# Autodesk Inventor assembly: populated-keyboard_cherrymx
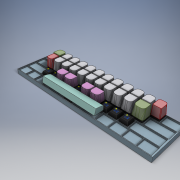
[picture p0: Inventor's stored thumbnail of the model, 180x180]
Saved by Autodesk Inventor 2016 (Build 200138000, 138)
## iProperties
Created: 2016-12-08
Part Number: populated-keyboard_cherrymx
Document SubType Name: Assembly
Designer: Cemra JC
Author: Cemra JC
## Documents named in this file (10)
- J:\The Files\The Software Files\Projects\stenotoppers\cherrymx\base-model\populated-keyboard_cherrymx.iam
- J:\The Files\The Software Files\Projects\stenotoppers\cherrymx\base-model\keyboard-mockup_cherrymx.iam
- J:\The Files\The Software Files\Projects\stenotoppers\cherrymx\base-model\standard-keycap_top-rows_base_cherrymx.ipt
- J:\The Files\The Software Files\Projects\stenotoppers\cherrymx\base-model\keyswitch_cherrymx.iam
- J:\The Files\The Software Files\Projects\stenotoppers\cherrymx\base-model\spacebar-keycap_mockup_cherrymx.ipt
- J:\The Files\The Software Files\Projects\stenotoppers\cherrymx\base-model\thumb-keycap_thumb-row_base_cherrymx.ipt
- J:\The Files\The Software Files\Projects\stenotoppers\cherrymx\base-model\standard-keycap_top-rows_base_cherrymx\smaller-keycap_top-rows_base_cherrymx.ipt
- J:\The Files\The Software Files\Projects\stenotoppers\cherrymx\base-model\standard-keycap_top-rows_base_cherrymx\larger-keycap_top-rows_base_cherrymx.ipt
- J:\The Files\The Software Files\Projects\stenotoppers\cherrymx\base-model\standard-keycap_top-rows_base_cherrymx\standard-keycap_top-rows_base_cherrymx.ipt
- J:\The Files\The Software Files\Projects\stenotoppers\parameters.xlsx
## Components (30 placed, 7 different names)
1. keyboard-mockup_cherrymx:1 [sub-assembly] — Rigid:5, Rigid:11, Rigid:12, Rigid:13, Rigid:14, Rigid:15, Rigid:16, Rigid:17, Rigid:18
2. keyswitch_cherrymx:1 [sub-assembly] — Rigid:5, Rigid:10
3. spacebar-keycap_mockup_cherrymx:1 — Rigid:10
4. smaller-keycap_top-rows_base_cherrymx:1 — Rigid:13
5. smaller-keycap_top-rows_base_cherrymx:2 — Rigid:16
6. larger-keycap_top-rows_base_cherrymx:3 — Rigid:17
7. larger-keycap_top-rows_base_cherrymx:4 — Rigid:15
8. thumb-keycap_thumb-row_base_cherrymx:2 — Rigid:12
9. thumb-keycap_thumb-row_base_cherrymx:3
10. thumb-keycap_thumb-row_base_cherrymx:1 — Rigid:11
11. thumb-keycap_thumb-row_base_cherrymx:4
12. standard-keycap_top-rows_base_cherrymx:6 — Rigid:18
13. standard-keycap_top-rows_base_cherrymx:7
14. standard-keycap_top-rows_base_cherrymx:8
15. standard-keycap_top-rows_base_cherrymx:9
16. standard-keycap_top-rows_base_cherrymx:10
17. standard-keycap_top-rows_base_cherrymx:11
18. standard-keycap_top-rows_base_cherrymx:12
19. standard-keycap_top-rows_base_cherrymx:13
20. standard-keycap_top-rows_base_cherrymx:14
21. standard-keycap_top-rows_base_cherrymx:15
22. standard-keycap_top-rows_base_cherrymx:5 — Rigid:14
23. standard-keycap_top-rows_base_cherrymx:16
24. standard-keycap_top-rows_base_cherrymx:17
25. standard-keycap_top-rows_base_cherrymx:18
26. standard-keycap_top-rows_base_cherrymx:19
27. standard-keycap_top-rows_base_cherrymx:20
28. standard-keycap_top-rows_base_cherrymx:21
29. standard-keycap_top-rows_base_cherrymx:22
30. standard-keycap_top-rows_base_cherrymx:23
## Component patterns: (2 elements, first: thumb-keycap_thumb-row_base_cherrymx:2), (2 elements, first: thumb-keycap_thumb-row_base_cherrymx:1), (10 elements, first: standard-keycap_top-rows_base_cherrymx:6), (9 elements, first: standard-keycap_top-rows_base_cherrymx:5)
## Relationships (10: WeldJoint 10)
- Rigid:5 [WeldJoint]: keyboard-mockup_cherrymx:1 ↔ keyswitch_cherrymx:1
- Rigid:10 [WeldJoint]: keyswitch_cherrymx:1 ↔ spacebar-keycap_mockup_cherrymx:1
- Rigid:11 [WeldJoint]: keyboard-mockup_cherrymx:1 ↔ thumb-keycap_thumb-row_base_cherrymx:1
- Rigid:12 [WeldJoint]: keyboard-mockup_cherrymx:1 ↔ thumb-keycap_thumb-row_base_cherrymx:2
- Rigid:13 [WeldJoint]: keyboard-mockup_cherrymx:1 ↔ smaller-keycap_top-rows_base_cherrymx:1
- Rigid:14 [WeldJoint]: keyboard-mockup_cherrymx:1 ↔ standard-keycap_top-rows_base_cherrymx:5
- Rigid:15 [WeldJoint]: keyboard-mockup_cherrymx:1 ↔ larger-keycap_top-rows_base_cherrymx:4
- Rigid:16 [WeldJoint]: keyboard-mockup_cherrymx:1 ↔ smaller-keycap_top-rows_base_cherrymx:2
- Rigid:17 [WeldJoint]: keyboard-mockup_cherrymx:1 ↔ larger-keycap_top-rows_base_cherrymx:3
- Rigid:18 [WeldJoint]: keyboard-mockup_cherrymx:1 ↔ standard-keycap_top-rows_base_cherrymx:6
## Named parameters: k_width = 18.1 mm, k_height = 18 mm, k_height_t = 16 mm, k_taper1 = 1.5 mm, k_taper2 = 0.5 mm, k_staper = 1 mm, k_sradius = 4 mm, k_ltaper = 1.5 mm, k_lradius = 6 mm, k_radius = 6 mm, k_wthick = 1.5 mm, k_ribthick = 1.5 mm, k_ribheight = 5 mm, k_poleoff = 2.2625 mm, k_poledia = 5.54 mm, k_cmxw = 1.35 mm, k_cmxl = 4.4 mm, s_bwidth = 15.6 mm, s_poleh = 3.6 mm, s_polebw = 5.5 mm, s_polebl = 7 mm, b_pad = 1 mm, b_tab = 27.15 mm, b_caps = 31.675 mm, b_lshift = 40.725 mm, b_rshift = 49.775 mm, b_ctrl = 22.625 mm, b_space = 117.65 mm, b_width = 286.5 mm, b_height = 77.4 mm
